# Autodesk Inventor assembly: Assembly6
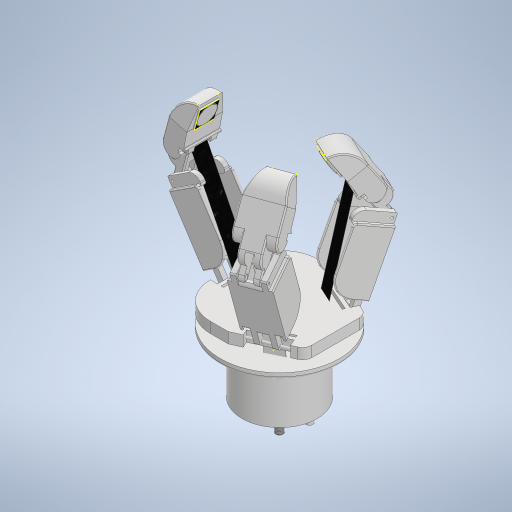
[picture p0: Inventor's stored thumbnail of the model, 512x512]
Saved by Autodesk Inventor 2024.3 (Build 283343000, 343)
## iProperties
Created: 2024-11-16
Part Number: Assembly6
Document SubType Name: Assembly
Designer: Ryba
Author: Ryba
## Documents named in this file (11)
- C:\Users\Ryba\Desktop\GRIPPERRRRR\Assembly6.iam
- C:\Users\Ryba\Desktop\GRIPPERRRRR\finger1.ipt
- C:\Users\Ryba\Desktop\GRIPPERRRRR\finger2.ipt
- C:\Users\Ryba\Desktop\GRIPPERRRRR\palm.ipt
- C:\Users\Ryba\Desktop\GRIPPERRRRR\platform.ipt
- C:\Users\Ryba\Desktop\GRIPPERRRRR\BELT.ipt
- C:\Users\Ryba\Desktop\GRIPPERRRRR\Part140.ipt
- C:\Users\Ryba\Desktop\GRIPPERRRRR\rubber.ipt
- C:\Users\Ryba\Desktop\GRIPPERRRRR\palmPlatform.ipt
- C:\Users\Ryba\Desktop\GRIPPERRRRR\distanceSensor.ipt
- C:\Users\Ryba\Desktop\GRIPPERRRRR\touchingSensor.ipt
## Components (20 placed, 10 different names)
1. finger1:1
2. finger2:1
3. palm:1
4. platform:1 — Cylindrical:1
5. finger1:2
6. finger2:2
7. finger1:3 — Mate:1, Mate:2
8. finger2:3
9. BELT:1 — Mate:1, Mate:2
10. BELT:2
11. BELT:3
12. Part140:1
13. rubber:1
14. rubber:2
15. rubber:3
16. palmPlatform:1 — Cylindrical:1
17. distanceSensor:1
18. touchingSensor:1
19. touchingSensor:2
20. touchingSensor:3
## Relationships (3: Mate 2, CylindricalJoint 1)
- Mate:1: finger1:3 ↔ BELT:1
- Mate:2: finger1:3 ↔ BELT:1
- Cylindrical:1: platform:1 ↔ palmPlatform:1
## Named parameters: Finish1_Area = 54.98
note: some values were not read from the file. Shown as the stored number, unit unknown: "Finish1_Area".
